# Autodesk Inventor assembly: Assembly_Trial_2
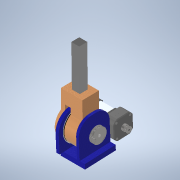
[picture p0: Inventor's stored thumbnail of the model, 180x180]
Saved by Autodesk Inventor 2022 (Build 260153000, 153)
## iProperties
Created: 2022-01-01
Part Number: Assembly_Trial_2
Document SubType Name: Assembly
Designer: Mlees
Author: Mlees
## Documents named in this file (18)
- F:\404 Engineering Arm\Assembly_Trial_2.iam
- F:\404 Engineering Arm\Downloaded Parts\nema17-speed-reducer-1.snapshot.9\24_Teeth_Sun_Gear.step.ipt
- F:\404 Engineering Arm\Downloaded Parts\nema17-speed-reducer-1.snapshot.9\36_Teeth_Planet_Gear.step.ipt
- F:\404 Engineering Arm\Downloaded Parts\nema17-speed-reducer-1.snapshot.9\96_Teeth_Gear.step.ipt
- F:\404 Engineering Arm\Downloaded Parts\nema17-speed-reducer-1.snapshot.9\Gear_Cover.ipt
- F:\404 Engineering Arm\Downloaded Parts\nema17-speed-reducer-1.snapshot.9\Plamet_Carrier.ipt
- F:\404 Engineering Arm\Downloaded Parts\Nema17-115oz-in-holding\stp-mtr-17060w.ipt
- F:\404 Engineering Arm\Downloaded Parts\nema-17-motor-mount-1.snapshot.1\NEMA_17_Bracket.ipt
- F:\404 Engineering Arm\Downloaded Parts\Pully_System\GT2 20T Drive Pulley.ipt
- F:\404 Engineering Arm\Downloaded Parts\Pully_System\GT2 60T Drive Pulley.ipt
- F:\404 Engineering Arm\Downloaded Parts\75mm_Harmonic_Drive\Radial Bearings\6815 bearing.ipt
- F:\404 Engineering Arm\Created Parts\Base.ipt
- F:\404 Engineering Arm\Created Parts\Harmonic Drive Mount.ipt
- F:\404 Engineering Arm\Downloaded Parts\75mm_Harmonic_Drive\HarmonicDrive75mmV2.iam
- F:\404 Engineering Arm\Created Parts\Base_Attachment.ipt
- F:\404 Engineering Arm\Created Parts\DriveShaft.ipt
- F:\404 Engineering Arm\Created Parts\Tilt_Portion.ipt
- F:\404 Engineering Arm\Created Parts\Attachment_Shaft.ipt
## Components (19 placed, 17 different names)
1. 24_Teeth_Sun_Gear.step:1 — Rotational:1, Rotational:5
2. 36_Teeth_Planet_Gear.step:1 — Rotational:2
3. 96_Teeth_Gear.step:1 — Rigid:2, Rigid:3
4. Gear_Cover:1 — Rigid:3
5. Plamet_Carrier:1 — Rotational:2, Rotational:3, Rotational:4, Rotational:5, Rotational:6
6. stp-mtr-17060w:1 — Rigid:1, Rotational:1
7. NEMA_17_Bracket:1 — Rigid:1, Rigid:2, Rigid:4
8. GT2 20T Drive Pulley:1 — Rotational:6
9. GT2 60T Drive Pulley:1 — Rotational:9, Rigid:7
10. 6815 bearing:1 — Rotational:7, Rotational:8
11. Harmonic Drive Mount:1 — Rotational:8, Rigid:5, Rigid:6
12. 36_Teeth_Planet_Gear.step:2 — Rotational:3
13. 36_Teeth_Planet_Gear.step:3 — Rotational:4
14. Base:1 — Rigid:4, Rigid:5
15. HarmonicDrive75mmV2:1 [sub-assembly] — Rotational:7, Rotational:10
16. Base_Attachment:1 — Rigid:6, Rotational:9
17. DriveShaft:1 — Rigid:7
18. Tilt_Portion:1 — Rotational:10, Rigid:8
19. Attachment_Shaft:1 — Rigid:8
## Relationships (18: RevoluteJoint 10, WeldJoint 8)
- Rigid:1 [WeldJoint]: stp-mtr-17060w:1 ↔ NEMA_17_Bracket:1
- Rigid:2 [WeldJoint]: 96_Teeth_Gear.step:1 ↔ NEMA_17_Bracket:1
- Rotational:1 [RevoluteJoint]: 24_Teeth_Sun_Gear.step:1 ↔ stp-mtr-17060w:1
- Rotational:2 [RevoluteJoint]: 36_Teeth_Planet_Gear.step:1 ↔ Plamet_Carrier:1
- Rotational:3 [RevoluteJoint]: Plamet_Carrier:1 ↔ 36_Teeth_Planet_Gear.step:2
- Rotational:4 [RevoluteJoint]: Plamet_Carrier:1 ↔ 36_Teeth_Planet_Gear.step:3
- Rotational:5 [RevoluteJoint]: 24_Teeth_Sun_Gear.step:1 ↔ Plamet_Carrier:1
- Rigid:3 [WeldJoint]: 96_Teeth_Gear.step:1 ↔ Gear_Cover:1
- Rigid:4 [WeldJoint]: NEMA_17_Bracket:1 ↔ Base:1
- Rotational:6 [RevoluteJoint]: Plamet_Carrier:1 ↔ GT2 20T Drive Pulley:1
- Rotational:7 [RevoluteJoint]: 6815 bearing:1 ↔ HarmonicDrive75mmV2:1
- Rotational:8 [RevoluteJoint]: 6815 bearing:1 ↔ Harmonic Drive Mount:1
- Rigid:5 [WeldJoint]: Harmonic Drive Mount:1 ↔ Base:1
- Rigid:6 [WeldJoint]: Harmonic Drive Mount:1 ↔ Base_Attachment:1
- Rotational:9 [RevoluteJoint]: GT2 60T Drive Pulley:1 ↔ Base_Attachment:1
- Rigid:7 [WeldJoint]: GT2 60T Drive Pulley:1 ↔ DriveShaft:1
- Rotational:10 [RevoluteJoint]: HarmonicDrive75mmV2:1 ↔ Tilt_Portion:1
- Rigid:8 [WeldJoint]: Tilt_Portion:1 ↔ Attachment_Shaft:1
